# Autodesk Inventor assembly: Assembly
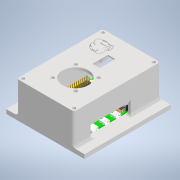
[picture p0: Inventor's stored thumbnail of the model, 180x180]
Saved by Autodesk Inventor 2020 (Build 240168000, 168)
## iProperties
Created: 2020-01-18
Part Number: Assembly
Document SubType Name: Assembly
Designer: chris
Author: chris
## Documents named in this file (4)
- C:\Users\Chris Gerth\Documents\Robotics\RobotCasserole2020\piVisionCase\Assembly.iam
- C:\Users\Chris Gerth\Documents\Robotics\RobotCasserole2020\piVisionCase\Raspberry Pi 4 Model B.iam
- C:\Users\Chris Gerth\Documents\Robotics\RobotCasserole2020\piVisionCase\bottom.ipt
- C:\Users\Chris Gerth\Documents\Robotics\RobotCasserole2020\piVisionCase\top.ipt
## Components (3 placed, 3 different names)
1. Raspberry Pi 4 Model B:1 [sub-assembly] — Insert:1, Angle:1
2. bottom:1 — Insert:1, Angle:1, Mate:1, Flush:1
3. top:1 — Mate:1, Flush:1
## Relationships (4: Insert 1, Angle 1, Mate 1, Flush 1)
- Insert:1: Raspberry Pi 4 Model B:1 ↔ bottom:1
- Angle:1 (180 deg): Raspberry Pi 4 Model B:1 ↔ bottom:1
- Mate:1: bottom:1 ↔ top:1
- Flush:1: bottom:1 ↔ top:1
